# Autodesk Inventor assembly: 100-10-FRAME-DIFFERENTIAL-REINF-01
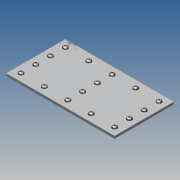
[picture p0: Inventor's stored thumbnail of the model, 180x180]
Saved by Autodesk Inventor 2018.2 (Build 222227000, 227)
## iProperties
Manager: feesmrt
Company: FRANCOR
Part Number: 100-10-FRAME-DIFFERENTIAL-REINF-01
Project: Rescue Robot
Cost Center: -
Material: Generisch
Document SubType Name: Assembly
Designer: feesmrt
Engineer: feesmrt
Authority: feesmrt
Description: Verbinder Differential Verstärkungsblech
Stock Number: 100-10-FRAME-DIFFERENTIAL-REINF-02
Subject: Rescue Robot
Author: feesmrt
Revision Number: 1
Title: Verbinder Differential Verstärkungsblech
## Documents named in this file (3)
- C:\Users\feesmrt\Documents\FRANC0R\CAD\02-Rocker-Bogie-Robot\100-CHASSIS\10-FRAME\100-10-FRAME-DIFFERENTIAL-REINF-01.iam
- C:\Users\feesmrt\Documents\FRANC0R\CAD\02-Rocker-Bogie-Robot\100-CHASSIS\10-FRAME\100-10-FRAME-DIFFERENTIAL-REINF-01.ipt
- C:\Users\feesmrt\Documents\FRANC0R\CAD\02-Rocker-Bogie-Robot\100-CHASSIS\10-FRAME\100-10-FRAME-DIFFERENTIAL-REINF-02.iam
## Components (17 placed, 2 different names)
1. 100-10-FRAME-DIFFERENTIAL-REINF-01:1 — Passend:1, Passend:2, Winkel:1, Passend:4, Passend:5, Winkel:2, Passend:6, Passend:7, Winkel:3
2. 100-10-FRAME-DIFFERENTIAL-REINF-02:1 [sub-assembly] — Passend:1, Passend:2, Winkel:1
3. 100-10-FRAME-DIFFERENTIAL-REINF-02:2 [sub-assembly]
4. 100-10-FRAME-DIFFERENTIAL-REINF-02:3 [sub-assembly]
5. 100-10-FRAME-DIFFERENTIAL-REINF-02:4 [sub-assembly]
6. 100-10-FRAME-DIFFERENTIAL-REINF-02:5 [sub-assembly]
7. 100-10-FRAME-DIFFERENTIAL-REINF-02:6 [sub-assembly]
8. 100-10-FRAME-DIFFERENTIAL-REINF-02:7 [sub-assembly]
9. 100-10-FRAME-DIFFERENTIAL-REINF-02:8 [sub-assembly]
10. 100-10-FRAME-DIFFERENTIAL-REINF-02:9 [sub-assembly]
11. 100-10-FRAME-DIFFERENTIAL-REINF-02:13 [sub-assembly] — Passend:4, Passend:5, Winkel:2
12. 100-10-FRAME-DIFFERENTIAL-REINF-02:14 [sub-assembly]
13. 100-10-FRAME-DIFFERENTIAL-REINF-02:15 [sub-assembly] — Passend:6, Passend:7, Winkel:3
14. 100-10-FRAME-DIFFERENTIAL-REINF-02:16 [sub-assembly]
15. 100-10-FRAME-DIFFERENTIAL-REINF-02:17 [sub-assembly]
16. 100-10-FRAME-DIFFERENTIAL-REINF-02:18 [sub-assembly]
17. 100-10-FRAME-DIFFERENTIAL-REINF-02:19 [sub-assembly]
## Component patterns: (9 elements, first: 100-10-FRAME-DIFFERENTIAL-REINF-02:1), (2 elements, first: 100-10-FRAME-DIFFERENTIAL-REINF-02:13), (5 elements, first: 100-10-FRAME-DIFFERENTIAL-REINF-02:15)
## Relationships (9: Mate 6, Angle 3)
- Passend:1 [Mate]: 100-10-FRAME-DIFFERENTIAL-REINF-01:1 ↔ 100-10-FRAME-DIFFERENTIAL-REINF-02:1
- Passend:2 [Mate]: 100-10-FRAME-DIFFERENTIAL-REINF-01:1 ↔ 100-10-FRAME-DIFFERENTIAL-REINF-02:1
- Winkel:1 [Angle] (0 deg): 100-10-FRAME-DIFFERENTIAL-REINF-01:1 ↔ 100-10-FRAME-DIFFERENTIAL-REINF-02:1
- Passend:4 [Mate]: 100-10-FRAME-DIFFERENTIAL-REINF-01:1 ↔ 100-10-FRAME-DIFFERENTIAL-REINF-02:13
- Passend:5 [Mate] (2.8 mm): 100-10-FRAME-DIFFERENTIAL-REINF-01:1 ↔ 100-10-FRAME-DIFFERENTIAL-REINF-02:13
- Winkel:2 [Angle] (0 deg): 100-10-FRAME-DIFFERENTIAL-REINF-01:1 ↔ 100-10-FRAME-DIFFERENTIAL-REINF-02:13
- Passend:6 [Mate]: 100-10-FRAME-DIFFERENTIAL-REINF-01:1 ↔ 100-10-FRAME-DIFFERENTIAL-REINF-02:15
- Passend:7 [Mate]: 100-10-FRAME-DIFFERENTIAL-REINF-01:1 ↔ 100-10-FRAME-DIFFERENTIAL-REINF-02:15
- Winkel:3 [Angle] (0 deg): 100-10-FRAME-DIFFERENTIAL-REINF-01:1 ↔ 100-10-FRAME-DIFFERENTIAL-REINF-02:15
